# Autodesk Inventor assembly: plateaumonte6GV2202
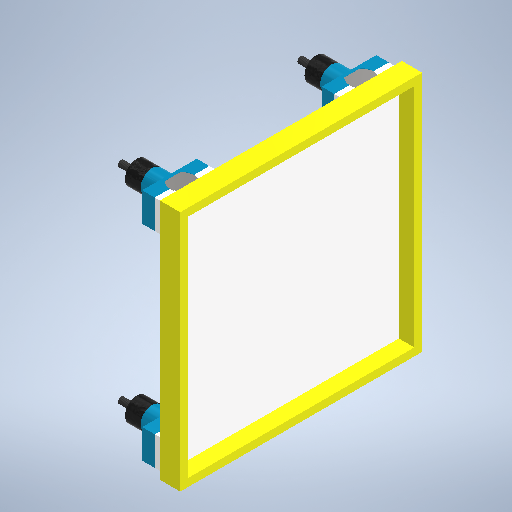
[picture p0: Inventor's stored thumbnail of the model, 512x512]
Saved by Autodesk Inventor 2025.2 (Build 292293000, 293)
## iProperties
Created: 2025-02-21
Part Number: plateaumonte6GV2202
Document SubType Name: Assembly
Designer: antoi
Author: antoi
## Documents named in this file (6)
- C:\Users\antoi\Documents\Henallux_24_25\Q2\proj\prototype\plateaumonte6GV2202.iam
- C:\Users\antoi\Documents\Henallux_24_25\Q2\proj\prototype\moteurG6V2.ipt
- C:\Users\antoi\Documents\Henallux_24_25\Q2\proj\prototype\plateauV2102.ipt
- C:\Users\antoi\Documents\Henallux_24_25\Q2\proj\prototype\bagueSilentbloc.ipt
- C:\Users\antoi\Documents\Henallux_24_25\Q2\proj\prototype\rebord1515.ipt
- C:\Users\antoi\Documents\Henallux_24_25\Q2\proj\prototype\silentBloc.ipt
## Components (14 placed, 5 different names)
1. plateauV2102:1 — Placage:1, Affleurement:1, Affleurement:2, Affleurement:3, Placage:3, Placage:4, Placage:5
2. rebord1515:1 — Placage:3, Placage:4, Placage:5
3. moteurG6V2:1 — Placage:1, Affleurement:1
4. moteurG6V2:2 — Placage:2
5. moteurG6V2:3
6. moteurG6V2:4
7. bagueSilentbloc:1 — Placage:2, Affleurement:2, Affleurement:3
8. bagueSilentbloc:2 — Placage:6, Placage:7
9. bagueSilentbloc:3
10. bagueSilentbloc:4
11. silentBloc:1 — Placage:6, Placage:7
12. silentBloc:2
13. silentBloc:3
14. silentBloc:4
## Component patterns: (4 elements, first: moteurG6V2:1), (4 elements, first: bagueSilentbloc:1), (4 elements, first: silentBloc:1)
## Relationships (10: Mate 7, Flush 3)
- Placage:1 [Mate]: plateauV2102:1 ↔ moteurG6V2:1
- Affleurement:1 [Flush]: plateauV2102:1 ↔ moteurG6V2:1
- Placage:2 [Mate]: moteurG6V2:2 ↔ bagueSilentbloc:1
- Affleurement:2 [Flush]: plateauV2102:1 ↔ bagueSilentbloc:1
- Affleurement:3 [Flush]: plateauV2102:1 ↔ bagueSilentbloc:1
- Placage:3 [Mate]: plateauV2102:1 ↔ rebord1515:1
- Placage:4 [Mate]: plateauV2102:1 ↔ rebord1515:1
- Placage:5 [Mate]: plateauV2102:1 ↔ rebord1515:1
- Placage:6 [Mate]: bagueSilentbloc:2 ↔ silentBloc:1
- Placage:7 [Mate]: bagueSilentbloc:2 ↔ silentBloc:1
